# Autodesk Inventor assembly: PivotAssembly
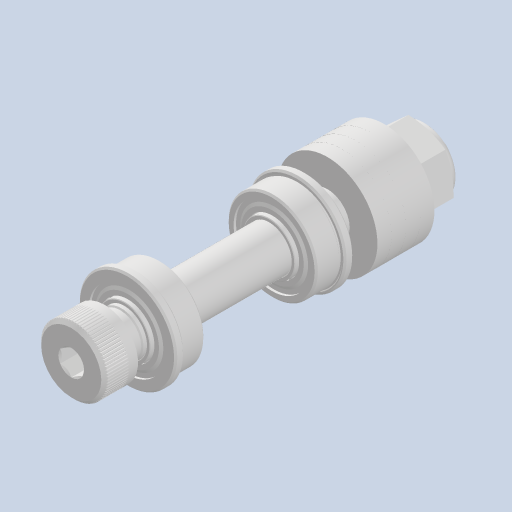
[picture p0: Inventor's stored thumbnail of the model, 512x512]
Saved by Autodesk Inventor 2023 (Build 270158000, 158)
## iProperties
Created: 2023-03-28
Part Number: PivotAssembly
Document SubType Name: Assembly
Designer: Dave
Author: Dave
## Documents named in this file (5)
- C:\Users\megan\OneDrive\Documents\GitHub\BehrendURCMechanical\CAD\Chassis V3\Pivot Files and Assembly\PivotAssembly.iam
- C:\Users\megan\OneDrive\Documents\GitHub\BehrendURCMechanical\CAD\Chassis V3\Pivot Files and Assembly\57155K337_Stainless Steel Ball Bearing1.ipt
- C:\Users\megan\OneDrive\Documents\GitHub\BehrendURCMechanical\CAD\Chassis V3\Pivot Files and Assembly\91259A546_Alloy Steel Shoulder Screw1.ipt
- C:\Users\megan\OneDrive\Documents\GitHub\BehrendURCMechanical\CAD\Chassis V3\Pivot Files and Assembly\91831A011_18-8 Stainless Steel Nylon-Insert Locknut (1).ipt
- C:\Users\megan\OneDrive\Documents\GitHub\BehrendURCMechanical\CAD\Chassis V3\Pivot Files and Assembly\96659A105_18-8 Stainless Steel SAE Washer1.ipt
## Components (8 placed, 4 different names)
1. 57155K337_Stainless Steel Ball Bearing1:1 — Mate:3, Mate:4, Mate:6
2. 91259A546_Alloy Steel Shoulder Screw1:1 — Mate:1, Mate:2, Mate:3, Mate:5, Mate:8, Mate:10, Mate:12, Mate:13
3. 91831A011_18-8 Stainless Steel Nylon-Insert Locknut (1):1 — Mate:13, Mate:14
4. 57155K337_Stainless Steel Ball Bearing1:2 — Mate:1, Mate:2, Mate:4
5. 96659A105_18-8 Stainless Steel SAE Washer1:1 — Mate:7, Mate:8, Mate:9
6. 96659A105_18-8 Stainless Steel SAE Washer1:2 — Mate:5, Mate:6, Mate:7
7. 96659A105_18-8 Stainless Steel SAE Washer1:3 — Mate:9, Mate:10, Mate:11
8. 96659A105_18-8 Stainless Steel SAE Washer1:4 — Mate:11, Mate:12, Mate:14
## Relationships (14: Mate 14)
- Mate:1: 91259A546_Alloy Steel Shoulder Screw1:1 ↔ 57155K337_Stainless Steel Ball Bearing1:2
- Mate:2 (3.175 mm): 91259A546_Alloy Steel Shoulder Screw1:1 ↔ 57155K337_Stainless Steel Ball Bearing1:2
- Mate:3: 57155K337_Stainless Steel Ball Bearing1:1 ↔ 91259A546_Alloy Steel Shoulder Screw1:1
- Mate:4 (-25.4 mm): 57155K337_Stainless Steel Ball Bearing1:1 ↔ 57155K337_Stainless Steel Ball Bearing1:2
- Mate:5: 91259A546_Alloy Steel Shoulder Screw1:1 ↔ 96659A105_18-8 Stainless Steel SAE Washer1:2
- Mate:6 (3.175 mm): 57155K337_Stainless Steel Ball Bearing1:1 ↔ 96659A105_18-8 Stainless Steel SAE Washer1:2
- Mate:7: 96659A105_18-8 Stainless Steel SAE Washer1:1 ↔ 96659A105_18-8 Stainless Steel SAE Washer1:2
- Mate:8: 91259A546_Alloy Steel Shoulder Screw1:1 ↔ 96659A105_18-8 Stainless Steel SAE Washer1:1
- Mate:9: 96659A105_18-8 Stainless Steel SAE Washer1:1 ↔ 96659A105_18-8 Stainless Steel SAE Washer1:3
- Mate:10: 91259A546_Alloy Steel Shoulder Screw1:1 ↔ 96659A105_18-8 Stainless Steel SAE Washer1:3
- Mate:11: 96659A105_18-8 Stainless Steel SAE Washer1:3 ↔ 96659A105_18-8 Stainless Steel SAE Washer1:4
- Mate:12: 91259A546_Alloy Steel Shoulder Screw1:1 ↔ 96659A105_18-8 Stainless Steel SAE Washer1:4
- Mate:13: 91259A546_Alloy Steel Shoulder Screw1:1 ↔ 91831A011_18-8 Stainless Steel Nylon-Insert Locknut (1):1
- Mate:14: 91831A011_18-8 Stainless Steel Nylon-Insert Locknut (1):1 ↔ 96659A105_18-8 Stainless Steel SAE Washer1:4
